# Autodesk Inventor assembly: Aimbot_Rev2
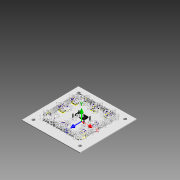
[picture p0: Inventor's stored thumbnail of the model, 180x180]
Saved by Autodesk Inventor 2015 (Build 190159000, 159)
## iProperties
Manager: Swagfish
Company: AntiWaseem Industries (AWI)
Created: 2014-05-17
Part Number: Aimbot_Rev2
Document SubType Name: Assembly
Designer: Joseph Varikooty
Mass: 2661.26 g
Surface Area: 7608.41 cm^2
Volume: 1160.78 cm^3
Density: 2.29266 g/cm^3
Author: Joseph Varikooty
Title: Aimbot Rev1.0
Subject: Rezzonating Swag
## Documents named in this file (97)
- X:\Dropbox\_School\AimBot\Aimbot_Rev2.iam
- X:\Dropbox\_School\AimBot\U-Channel Housing 4x2x12.ipt
- X:\Dropbox\_School\AimBot\HS-7940TH Servo.iam
- X:\Dropbox\_School\AimBot\Standard Servo Plate A (575112).ipt
- X:\Dropbox\_School\AimBot\Steel Ball Bearing (6383K245).iam
- X:\Dropbox\_School\AimBot\Turntable (1544T1).iam
- X:\Dropbox\_School\AimBot\Round Base A (585438).ipt
- X:\Dropbox\_School\AimBot\Bore Tube Clamp Hub (545340).ipt
- X:\Dropbox\_School\AimBot\Servo Hub - Tall (Hitec Standard) (ROB-12227).ipt
- X:\Dropbox\_School\AimBot\U Arms.ipt
- X:\Dropbox\_School\AimBot\Assembly1\Design Accelerator\Bolted Connection1.iam
- X:\Dropbox\_School\AimBot\Assembly1\Design Accelerator\Bolted Connection2.iam
- X:\Dropbox\_School\AimBot\Assembly1\Design Accelerator\Bolted Connection3.iam
- X:\Dropbox\_School\AimBot\Assembly1\Design Accelerator\Bolted Connection4.iam
- X:\Dropbox\_School\AimBot\Assembly1\Design Accelerator\Bolted Connection5.iam
- X:\Dropbox\_School\AimBot\Assembly1\Design Accelerator\Bolted Connection6.iam
- X:\Dropbox\_School\AimBot\Assembly1\Design Accelerator\Bolted Connection7.iam
- X:\Dropbox\_School\AimBot\Assembly1\Design Accelerator\Bolted Connection8.iam
- X:\Dropbox\_School\AimBot\Assembly1\Design Accelerator\Bolted Connection9.iam
- X:\Dropbox\_School\AimBot\Assembly1\Design Accelerator\Bolted Connection10.iam
- X:\Dropbox\_School\AimBot\Assembly1\Design Accelerator\Bolted Connection11.iam
- X:\Dropbox\_School\AimBot\Assembly1\Design Accelerator\Bolted Connection12.iam
- X:\Dropbox\_School\AimBot\Assembly1\Design Accelerator\Bolted Connection13.iam
- X:\Dropbox\_School\AimBot\64T Gear.ipt
- X:\Dropbox\_School\AimBot\32T Pinion Gear.ipt
- X:\Dropbox\_School\AimBot\Axail Rod.ipt
- X:\Dropbox\_School\AimBot\Spacer_ServoTilitBracketArm.ipt
- X:\Dropbox\_School\AimBot\Assembly1\Design Accelerator\Bolted Connection14.iam
- X:\Dropbox\_School\AimBot\Assembly1\Design Accelerator\Bolted Connection15.iam
- X:\Dropbox\_School\AimBot\Assembly1\Design Accelerator\Bolted Connection16.iam
- X:\Dropbox\_School\AimBot\Assembly1\Design Accelerator\Bolted Connection17.iam
- X:\Dropbox\_School\AimBot\Standoff_ServoTilitGearHub.ipt
- X:\Dropbox\_School\AimBot\Assembly1\Design Accelerator\Bolted Connection18.iam
- X:\Dropbox\_School\AimBot\Assembly1\Design Accelerator\Bolted Connection19.iam
- X:\Dropbox\_School\AimBot\Assembly1\Design Accelerator\Bolted Connection20.iam
- X:\Dropbox\_School\AimBot\Assembly1\Design Accelerator\Bolted Connection21.iam
- X:\Dropbox\_School\AimBot\Assembly1\Design Accelerator\Bolted Connection22.iam
- X:\Dropbox\_School\AimBot\Assembly1\Design Accelerator\Bolted Connection23.iam
- X:\Dropbox\_School\AimBot\Assembly1\Design Accelerator\Bolted Connection24.iam
- X:\Dropbox\_School\AimBot\Assembly1\Design Accelerator\Bolted Connection25.iam
- X:\Dropbox\_School\AimBot\Assembly1\Design Accelerator\Bolted Connection26.iam
- X:\Dropbox\_School\AimBot\Assembly1\Design Accelerator\Bolted Connection27.iam
- X:\Dropbox\_School\AimBot\Assembly1\Design Accelerator\Bolted Connection28.iam
- X:\Dropbox\_School\AimBot\Assembly1\Design Accelerator\Bolted Connection29.iam
- X:\Dropbox\_School\AimBot\Assembly1\Design Accelerator\Bolted Connection30.iam
- X:\Dropbox\_School\AimBot\Assembly1\Design Accelerator\Bolted Connection31.iam
- X:\Dropbox\_School\AimBot\Assembly1\Design Accelerator\Bolted Connection32.iam
- X:\Dropbox\_School\AimBot\Assembly1\Design Accelerator\Bolted Connection33.iam
- X:\Dropbox\_School\AimBot\Assembly1\Design Accelerator\Bolted Connection34.iam
- X:\Dropbox\_School\AimBot\Assembly1\Design Accelerator\Bolted Connection35.iam
- X:\Dropbox\_School\AimBot\Assembly1\Design Accelerator\Bolted Connection36.iam
- X:\Dropbox\_School\AimBot\Assembly1\Design Accelerator\Bolted Connection37.iam
- X:\Dropbox\_School\AimBot\Assembly1\Design Accelerator\Bolted Connection38.iam
- X:\Dropbox\_School\AimBot\Assembly1\Design Accelerator\Bolted Connection39.iam
- X:\Dropbox\_School\AimBot\Assembly1\Design Accelerator\Bolted Connection40.iam
- X:\Dropbox\_School\AimBot\Assembly1\Design Accelerator\Bolted Connection41.iam
- X:\Dropbox\_School\AimBot\Standoff_ServoPanBasePlate.ipt
- X:\Dropbox\_School\AimBot\SealWasher.ipt
- X:\Dropbox\_School\AimBot\Assembly1\Design Accelerator\Bolted Connection54.iam
- X:\Dropbox\_School\AimBot\Assembly1\Design Accelerator\Bolted Connection55.iam
- X:\Dropbox\_School\AimBot\Assembly1\Design Accelerator\Bolted Connection56.iam
- X:\Dropbox\_School\AimBot\Assembly1\Design Accelerator\Bolted Connection57.iam
- X:\Dropbox\_School\AimBot\Assembly1\Design Accelerator\Bolted Connection58.iam
- X:\Dropbox\_School\AimBot\Assembly1\Design Accelerator\Bolted Connection59.iam
- X:\Dropbox\_School\AimBot\Assembly1\Design Accelerator\Bolted Connection60.iam
- X:\Dropbox\_School\AimBot\Assembly1\Design Accelerator\Bolted Connection61.iam
- X:\Dropbox\_School\AimBot\Assembly1\Design Accelerator\Bolted Connection62.iam
- X:\Dropbox\_School\AimBot\Assembly1\Design Accelerator\Bolted Connection63.iam
- X:\Dropbox\_School\AimBot\Assembly1\Design Accelerator\Bolted Connection64.iam
- X:\Dropbox\_School\AimBot\Assembly1\Design Accelerator\Bolted Connection65.iam
- X:\Dropbox\_School\AimBot\Assembly1\Design Accelerator\Bolted Connection66.iam
- X:\Dropbox\_School\AimBot\ODROID-XU+E.ipt
- X:\Dropbox\_School\AimBot\Assembly1\Design Accelerator\Bolted Connection67.iam
- X:\Dropbox\_School\AimBot\Assembly1\Design Accelerator\Bolted Connection68.iam
- X:\Dropbox\_School\AimBot\Assembly1\Design Accelerator\Bolted Connection69.iam
- X:\Dropbox\_School\AimBot\Assembly1\Design Accelerator\Bolted Connection70.iam
- X:\Dropbox\_School\AimBot\Bracket (15275A53).ipt
- X:\Dropbox\_School\AimBot\Base_Master_Rev2.ipt
- X:\Dropbox\_School\AimBot\BottomBasePlate_Rev2.ipt
- X:\Dropbox\_School\AimBot\Bracket (15275A53)_LeftCut.ipt
- X:\Dropbox\_School\AimBot\Aimbot_Rev2\Design Accelerator\Bolted Connection1.iam
- X:\Dropbox\_School\AimBot\Aimbot_Rev2\Design Accelerator\Bolted Connection2.iam
- X:\Dropbox\_School\AimBot\Aimbot_Rev2\Design Accelerator\Bolted Connection3.iam
- X:\Dropbox\_School\AimBot\Aimbot_Rev2\Design Accelerator\Bolted Connection4.iam
- X:\Dropbox\_School\AimBot\Aimbot_Rev2\Design Accelerator\Bolted Connection5.iam
- X:\Dropbox\_School\AimBot\Aimbot_Rev2\Design Accelerator\Bolted Connection6.iam
- X:\Dropbox\_School\AimBot\Aimbot_Rev2\Design Accelerator\Bolted Connection7.iam
- X:\Dropbox\_School\AimBot\Aimbot_Rev2\Design Accelerator\Bolted Connection8.iam
- X:\Dropbox\_School\AimBot\Aimbot_Rev2\Design Accelerator\Bolted Connection9.iam
- X:\Dropbox\_School\AimBot\Aimbot_Rev2\Design Accelerator\Bolted Connection10.iam
- X:\Dropbox\_School\AimBot\Aimbot_Rev2\Design Accelerator\Bolted Connection11.iam
- X:\Dropbox\_School\AimBot\Aimbot_Rev2\Design Accelerator\Bolted Connection12.iam
- X:\Dropbox\_School\AimBot\Aimbot_Rev2\Design Accelerator\Bolted Connection13.iam
- X:\Dropbox\_School\AimBot\Aimbot_Rev2\Design Accelerator\Bolted Connection14.iam
- X:\Dropbox\_School\AimBot\Aimbot_Rev2\Design Accelerator\Bolted Connection15.iam
- X:\Dropbox\_School\AimBot\Aimbot_Rev2\Design Accelerator\Bolted Connection16.iam
- X:\Dropbox\_School\AimBot\Aimbot_Rev2\Design Accelerator\Bolted Connection17.iam
## Components (133 placed, 22 different names)
1. U-Channel Housing 4x2x12:1 — Mate:4, Mate:5, Mate:6, Mate:7, Mate:8, Mate:9, Mate:26, Mate:27, Mate:28, Mate:29, Mate:30, Mate:31, Mate:32, Mate:33, Mate:34, Mate:35, Mate:36, Mate:37, Mate:38, Mate:39, Mate:40, Mate:41, Mate:42, Mate:43
2. HS-7940TH Servo:1 [sub-assembly] — RemoveAfterScrews:1, RemoveAfterScrews:2, Mate:46, Mate:47, Mate:48, Mate:50, Mate:51, Mate:52, Mate:219, Mate:221, Mate:223, Mate:225
3. Standard Servo Plate A (575112):1 — RemoveAfterScrews:1, RemoveAfterScrews:2, Mate:51, Mate:61, Mate:63, Mate:65, Mate:67, Mate:56, Mate:54, Mate:220, Mate:222, Mate:224, Mate:226
4. Steel Ball Bearing (6383K245):1 [sub-assembly] — Rigid:1, Cylindrical:2
5. Steel Ball Bearing (6383K245):2 [sub-assembly] — Rigid:2, Cylindrical:1, Flush:3
6. Turntable (1544T1):1 [sub-assembly] — Mate:10, Mate:11, Mate:12, Mate:136, Mate:137, Mate:138, Mate:139, Mate:140, Mate:141, Mate:143, Mate:145, Mate:147
7. Round Base A (585438):1 — Mate:21, BaseHub:22, BaseHub:23, BaseHub:24, BaseHub:25, BaseArm:97, BaseArm:98, BaseArm:99, BaseArm:100, Mate:101, Mate:109, Mate:111, Mate:113, Mate:115, Mate:117, Mate:119, Mate:121, Mate:123, Mate:125, Mate:127, Mate:129, Mate:131
8. Bore Tube Clamp Hub (545340):1 — Mate:7, Mate:8, Mate:9, Mate:45, Mate:69, Mate:70, Mate:71, Mate:72, Mate:73, Mate:74, Mate:75, Mate:76, Mate:80, Mate:89, Mate:90, Mate:91, Mate:92
9. Bore Tube Clamp Hub (545340):2 — Mate:4, Mate:5, Mate:6, Mate:44, Mate:93, Mate:94, Mate:95, Mate:96
10. Servo Hub - Tall (Hitec Standard) (ROB-12227):2 — Mate:21, BaseHub:22, BaseHub:23, BaseHub:24, BaseHub:25, Mate:134, Mate:135
11. HS-7940TH Servo:2 [sub-assembly] — Mate:3, Mate:132, Mate:133, Mate:134, Mate:135, Mate:227, Mate:229, Mate:231, Mate:233, Mate:235
12. Standard Servo Plate A (575112):2 — Mate:3, Mate:132, Mate:133, Angle:1, Mate:204, Mate:205, Mate:206, Mate:207, Mate:208, Mate:209, Mate:210, Mate:211, Mate:213, Mate:215, Mate:217, Mate:228, Mate:230, Mate:232, Mate:234, Mate:236
13. U Arms:1 — Rigid:1, Rigid:2, Mate:10, Mate:11, Mate:12, Mate:13, Mate:14, Mate:15, Mate:16, Mate:17, Mate:18, Mate:19, Mate:20, Mate:50, Mate:52, Mate:55, Mate:57, Mate:58, Mate:59, Mate:60, Mate:62, Mate:64, Mate:66, Mate:68, BaseArm:97, BaseArm:98, BaseArm:99, BaseArm:100, Mate:101, Mate:108, Mate:110, Mate:112, Mate:114, Mate:116, Mate:118, Mate:120, Mate:122, Mate:124, Mate:126, Mate:128, Mate:130
14. Bolted Connection:1 [sub-assembly] — Mate:13, Mate:14
15. Bolted Connection:2 [sub-assembly] — Mate:15, Mate:16
16. Bolted Connection:3 [sub-assembly] — Mate:17, Mate:18
17. Bolted Connection:4 [sub-assembly] — Mate:19, Mate:20
18. Bolted Connection:5 [sub-assembly] — Mate:26, Mate:27
19. Bolted Connection:6 [sub-assembly] — Mate:28, Mate:29
20. Bolted Connection:7 [sub-assembly] — Mate:30, Mate:31
21. Bolted Connection:8 [sub-assembly] — Mate:32, Mate:33
22. Bolted Connection:9 [sub-assembly] — Mate:34, Mate:35
23. Bolted Connection:10 [sub-assembly] — Mate:36, Mate:37
24. Bolted Connection:11 [sub-assembly] — Mate:38, Mate:39
25. Bolted Connection:12 [sub-assembly] — Mate:40, Mate:41
26. Bolted Connection:13 [sub-assembly] — Mate:42, Mate:43
27. 64T Gear:1 — Cylindrical:3, Rotation:1, Mate:79, Mate:80, Mate:81, Mate:82, Mate:83, Mate:84, Mate:85, Mate:86, Mate:87, Mate:88
28. 32T Pinion Gear:1 — Mate:46, Mate:47, Mate:48, Mate:49, Flush:2, Rotation:1
29. Axail Rod:1 — Cylindrical:1, Cylindrical:3, Mate:45, Mate:49, Flush:3
30. Axail Rod:2 — Cylindrical:2, Mate:44
31. Spacer_ServoTilitBracketArm:1 — Mate:53, Mate:54
32. Spacer_ServoTilitBracketArm:2 — Mate:55, Mate:56
33. Spacer_ServoTilitBracketArm:3 — Mate:57, Mate:58
34. Spacer_ServoTilitBracketArm:4 — Mate:59, Mate:60
35. Bolted Connection:14 [sub-assembly] — Mate:61, Mate:62
36. Bolted Connection:15 [sub-assembly] — Mate:63, Mate:64
37. Bolted Connection:16 [sub-assembly] — Mate:65, Mate:66
38. Bolted Connection:17 [sub-assembly] — Mate:67, Mate:68, Mate:53
39. Standoff_ServoTilitGearHub:1 — Mate:71, Mate:76, Mate:79
40. Standoff_ServoTilitGearHub:2 — Mate:70, Mate:74
41. Standoff_ServoTilitGearHub:3 — Mate:72, Mate:75
42. Standoff_ServoTilitGearHub:4 — Mate:69, Mate:73
43. Bolted Connection:18 [sub-assembly] — Mate:81, Mate:82
44. Bolted Connection:19 [sub-assembly] — Mate:83, Mate:84
45. Bolted Connection:20 [sub-assembly] — Mate:85, Mate:86
46. Bolted Connection:21 [sub-assembly] — Mate:87, Mate:88
47. Bolted Connection:22 [sub-assembly] — Mate:89, Mate:90
48. Bolted Connection:23 [sub-assembly] — Mate:91, Mate:92
49. Bolted Connection:24 [sub-assembly] — Mate:93, Mate:94
50. Bolted Connection:25 [sub-assembly] — Mate:95, Mate:96
51. Bolted Connection:26 [sub-assembly] — Mate:114, Mate:115
52. Bolted Connection:27 [sub-assembly] — Mate:112, Mate:113
53. Bolted Connection:28 [sub-assembly] — Mate:110, Mate:111
54. Bolted Connection:29 [sub-assembly] — Mate:108, Mate:109
55. Bolted Connection:30 [sub-assembly] — Mate:116, Mate:117
56. Bolted Connection:31 [sub-assembly] — Mate:118, Mate:119
57. Bolted Connection:32 [sub-assembly] — Mate:120, Mate:121
58. Bolted Connection:33 [sub-assembly] — Mate:122, Mate:123
59. Bolted Connection:34 [sub-assembly] — Mate:124, Mate:125
60. Bolted Connection:35 [sub-assembly] — Mate:126, Mate:127
61. Bolted Connection:36 [sub-assembly] — Mate:128, Mate:129
62. Bolted Connection:37 [sub-assembly] — Mate:130, Mate:131
63. BottomBasePlate_Rev2:1 — Mate:180, Mate:181, Mate:186, Mate:187, Mate:192, Mate:193, Mate:198, Mate:199, Angle:2, Mate:239, Mate:240, Mate:241, Mate:242, Mate:243, Mate:244, Mate:245, Mate:246, Mate:250, Mate:251, Mate:252, Mate:259, Mate:260, Mate:261, Mate:266, Mate:269, Mate:272, Mate:275, Mate:278, Mate:281, Mate:283, Mate:284, Mate:285, Mate:286, Mate:287, Mate:288, Mate:289, Mate:290, Mate:291, Mate:292, Mate:293, Mate:294, Mate:295, Mate:296, Mate:297, Mate:298, Mate:299, Mate:300, Mate:301, Mate:302, Mate:303, Mate:304
64. Base_Master_Rev2:1 — Mate:136, Mate:137, Mate:138, Mate:139, Mate:140, Mate:142, Mate:144, Mate:146, Mate:148, Angle:1, Mate:247, Mate:248, Mate:249, Mate:253, Mate:254, Mate:255, Mate:256, Mate:257, Mate:258, Mate:262, Mate:263, Mate:264, Mate:265, Mate:267, Mate:268, Mate:270, Mate:271, Mate:273, Mate:274, Mate:276, Mate:277, Mate:279, Mate:280, Mate:282, Mate:305, Mate:306, Mate:307, Mate:308, Mate:309, Mate:310, Mate:311, Mate:312, Mate:313, Mate:314, Mate:315, Mate:316
65. Bolted Connection:38 [sub-assembly] — Mate:141, Mate:142
66. Bolted Connection:39 [sub-assembly] — Mate:143, Mate:144
67. Bolted Connection:40 [sub-assembly] — Mate:145, Mate:146
68. Bolted Connection:41 [sub-assembly] — Mate:147, Mate:148
69. Standoff_ServoPanBasePlate:1 — Mate:200, Mate:205, Mate:207, Mate:214
70. Standoff_ServoPanBasePlate:2 — Mate:201, Mate:206, Mate:209, Mate:212
71. Standoff_ServoPanBasePlate:3 — Mate:203, Mate:210, Mate:216
72. Standoff_ServoPanBasePlate:4 — Mate:202, Mate:204, Mate:208, Mate:218
73. SealWasher:1 — Mate:189, Mate:191, Mate:202
74. SealWasher:2 — Mate:188, Mate:189, Mate:190, Mate:191
75. SealWasher:3 — Mate:188, Mate:190, Mate:192, Mate:193
76. SealWasher:4 — Mate:183, Mate:185, Mate:203
77. SealWasher:5 — Mate:182, Mate:183, Mate:184, Mate:186, Mate:187
78. SealWasher:6 — Mate:182, Mate:184, Mate:185
79. SealWasher:7 — Mate:177, Mate:178, Mate:201
80. SealWasher:8 — Mate:176, Mate:177, Mate:178, Mate:179
81. SealWasher:9 — Mate:176, Mate:179, Mate:180, Mate:181
82. SealWasher:10 — Mate:195, Mate:197, Mate:200
83. SealWasher:11 — Mate:194, Mate:195, Mate:196, Mate:197
84. SealWasher:12 — Mate:194, Mate:196, Mate:198, Mate:199
85. Bolted Connection:54 [sub-assembly] — Mate:211, Mate:212
86. Bolted Connection:55 [sub-assembly] — Mate:213, Mate:214
87. Bolted Connection:56 [sub-assembly] — Mate:215, Mate:216
88. Bolted Connection:57 [sub-assembly] — Mate:217, Mate:218
89. Bolted Connection:58 [sub-assembly] — Mate:219, Mate:220
90. Bolted Connection:59 [sub-assembly] — Mate:221, Mate:222
91. Bolted Connection:60 [sub-assembly] — Mate:223, Mate:224
92. Bolted Connection:61 [sub-assembly] — Mate:225, Mate:226
93. Bolted Connection:62 [sub-assembly] — Mate:227, Mate:228
94. Bolted Connection:63 [sub-assembly] — Mate:229, Mate:230
95. Bolted Connection:64 [sub-assembly] — Mate:231, Mate:232
96. Bolted Connection:65 [sub-assembly] — Mate:233, Mate:234
97. Bolted Connection:66 [sub-assembly] — Mate:235, Mate:236
98. ODROID-XU+E:1 — Angle:2
99. Bolted Connection:67 [sub-assembly] — Mate:241, Mate:242
100. Bolted Connection:68 [sub-assembly] — Mate:239, Mate:240
101. Bolted Connection:69 [sub-assembly] — Mate:243, Mate:244
102. Bolted Connection:70 [sub-assembly] — Mate:245, Mate:246
103. Bracket (15275A53):1 — Mate:249, Mate:252, Mate:253
104. Bracket (15275A53)_LeftCut:2 — Mate:247, Mate:250, Mate:255
105. Bracket (15275A53):3 — Mate:248, Mate:251, Mate:254
106. Bracket (15275A53)_LeftCut:3 — Mate:258, Mate:259, Mate:262
107. Bracket (15275A53):5 — Mate:256, Mate:261, Mate:264
108. Bracket (15275A53):6 — Mate:257, Mate:260, Mate:263
109. Bracket (15275A53):7 — Mate:268, Mate:269, Mate:270
110. Bracket (15275A53):8
111. Bracket (15275A53)_LeftCut:1 — Mate:265, Mate:266, Mate:267
112. Bracket (15275A53):9 — Mate:271, Mate:272, Mate:273
113. Bracket (15275A53):10
114. Bracket (15275A53):11 — Mate:274, Mate:275, Mate:276
115. Bracket (15275A53)_LeftCut:4 — Mate:280, Mate:281, Mate:282
116. Bracket (15275A53):13 — Mate:277, Mate:278, Mate:279
117. Bolted Connection:71 [sub-assembly] — Mate:283, Mate:284
118. Bolted Connection:72 [sub-assembly] — Mate:285, Mate:286
119. Bolted Connection:73 [sub-assembly] — Mate:287, Mate:288
120. Bolted Connection:74 [sub-assembly] — Mate:289, Mate:290
121. Bolted Connection:75 [sub-assembly] — Mate:291, Mate:292
122. Bolted Connection:76 [sub-assembly] — Mate:293, Mate:294
123. Bolted Connection:77 [sub-assembly] — Mate:295, Mate:296
124. Bolted Connection:78 [sub-assembly] — Mate:297, Mate:298
125. Bolted Connection:79 [sub-assembly] — Mate:299, Mate:300
126. Bolted Connection:80 [sub-assembly] — Mate:301, Mate:302
127. Bolted Connection:81 [sub-assembly] — Mate:303, Mate:304
128. Bolted Connection:82 [sub-assembly] — Mate:305, Mate:306
129. Bolted Connection:83 [sub-assembly] — Mate:307, Mate:308
130. Bolted Connection:84 [sub-assembly] — Mate:309, Mate:310
131. Bolted Connection:85 [sub-assembly] — Mate:311, Mate:312
132. Bolted Connection:86 [sub-assembly] — Mate:313, Mate:314
133. Bolted Connection:87 [sub-assembly] — Mate:315, Mate:316
## Relationships (289: Mate 279, CylindricalJoint 3, WeldJoint 2, Flush 2, Angle 2, RelateRotation 1)
- RemoveAfterScrews:1 [Mate]: HS-7940TH Servo:1 ↔ Standard Servo Plate A (575112):1
- RemoveAfterScrews:2 [Mate] (0.1651 mm): HS-7940TH Servo:1 ↔ Standard Servo Plate A (575112):1
- Mate:3 (0.1651 mm): HS-7940TH Servo:2 ↔ Standard Servo Plate A (575112):2
- Rigid:1 [WeldJoint]: Steel Ball Bearing (6383K245):1 ↔ U Arms:1
- Rigid:2 [WeldJoint]: Steel Ball Bearing (6383K245):2 ↔ U Arms:1
- Mate:4: U-Channel Housing 4x2x12:1 ↔ Bore Tube Clamp Hub (545340):2
- Mate:5: U-Channel Housing 4x2x12:1 ↔ Bore Tube Clamp Hub (545340):2
- Mate:6: U-Channel Housing 4x2x12:1 ↔ Bore Tube Clamp Hub (545340):2
- Mate:7: U-Channel Housing 4x2x12:1 ↔ Bore Tube Clamp Hub (545340):1
- Mate:8: U-Channel Housing 4x2x12:1 ↔ Bore Tube Clamp Hub (545340):1
- Mate:9: U-Channel Housing 4x2x12:1 ↔ Bore Tube Clamp Hub (545340):1
- Mate:10: Turntable (1544T1):1 ↔ U Arms:1
- Mate:11: Turntable (1544T1):1 ↔ U Arms:1
- Mate:12: Turntable (1544T1):1 ↔ U Arms:1
- Mate:13: U Arms:1 ↔ Bolted Connection:1
- Mate:14: U Arms:1 ↔ Bolted Connection:1
- Mate:15: U Arms:1 ↔ Bolted Connection:2
- Mate:16: U Arms:1 ↔ Bolted Connection:2
- Mate:17: U Arms:1 ↔ Bolted Connection:3
- Mate:18: U Arms:1 ↔ Bolted Connection:3
- Mate:19: U Arms:1 ↔ Bolted Connection:4
- Mate:20: U Arms:1 ↔ Bolted Connection:4
- Mate:21: Round Base A (585438):1 ↔ Servo Hub - Tall (Hitec Standard) (ROB-12227):2
- BaseHub:22 [Mate]: Round Base A (585438):1 ↔ Servo Hub - Tall (Hitec Standard) (ROB-12227):2
- BaseHub:23 [Mate]: Round Base A (585438):1 ↔ Servo Hub - Tall (Hitec Standard) (ROB-12227):2
- BaseHub:24 [Mate]: Round Base A (585438):1 ↔ Servo Hub - Tall (Hitec Standard) (ROB-12227):2
- BaseHub:25 [Mate]: Round Base A (585438):1 ↔ Servo Hub - Tall (Hitec Standard) (ROB-12227):2
- Mate:26: U-Channel Housing 4x2x12:1 ↔ Bolted Connection:5
- Mate:27: U-Channel Housing 4x2x12:1 ↔ Bolted Connection:5
- Mate:28: U-Channel Housing 4x2x12:1 ↔ Bolted Connection:6
- Mate:29: U-Channel Housing 4x2x12:1 ↔ Bolted Connection:6
- Mate:30: U-Channel Housing 4x2x12:1 ↔ Bolted Connection:7
- Mate:31: U-Channel Housing 4x2x12:1 ↔ Bolted Connection:7
- Mate:32: U-Channel Housing 4x2x12:1 ↔ Bolted Connection:8
- Mate:33: U-Channel Housing 4x2x12:1 ↔ Bolted Connection:8
- Mate:34: U-Channel Housing 4x2x12:1 ↔ Bolted Connection:9
- Mate:35: U-Channel Housing 4x2x12:1 ↔ Bolted Connection:9
- Mate:36: U-Channel Housing 4x2x12:1 ↔ Bolted Connection:10
- Mate:37: U-Channel Housing 4x2x12:1 ↔ Bolted Connection:10
- Mate:38: U-Channel Housing 4x2x12:1 ↔ Bolted Connection:11
- Mate:39: U-Channel Housing 4x2x12:1 ↔ Bolted Connection:11
- Mate:40: U-Channel Housing 4x2x12:1 ↔ Bolted Connection:12
- Mate:41: U-Channel Housing 4x2x12:1 ↔ Bolted Connection:12
- Mate:42: U-Channel Housing 4x2x12:1 ↔ Bolted Connection:13
- Mate:43: U-Channel Housing 4x2x12:1 ↔ Bolted Connection:13
- Cylindrical:1: Steel Ball Bearing (6383K245):2 ↔ Axail Rod:1
- Cylindrical:2: Steel Ball Bearing (6383K245):1 ↔ Axail Rod:2
- Cylindrical:3: 64T Gear:1 ↔ Axail Rod:1
- Mate:44: Bore Tube Clamp Hub (545340):2 ↔ Axail Rod:2
- Mate:45: Bore Tube Clamp Hub (545340):1 ↔ Axail Rod:1
- Mate:46: HS-7940TH Servo:1 ↔ 32T Pinion Gear:1
- Mate:47 (3.048 mm): HS-7940TH Servo:1 ↔ 32T Pinion Gear:1
- Mate:48: HS-7940TH Servo:1 ↔ 32T Pinion Gear:1
- Mate:49 (38.1 mm): 32T Pinion Gear:1 ↔ Axail Rod:1
- Flush:2: 32T Pinion Gear:1
- Rotation:1 [RelateRotation] (2 ul): 64T Gear:1 ↔ 32T Pinion Gear:1
- Mate:50: HS-7940TH Servo:1 ↔ U Arms:1
- Mate:51 (0.8255 mm): HS-7940TH Servo:1 ↔ Standard Servo Plate A (575112):1
- Mate:52: HS-7940TH Servo:1 ↔ U Arms:1
- Mate:53: Spacer_ServoTilitBracketArm:1 ↔ Bolted Connection:17
- Mate:54: Standard Servo Plate A (575112):1 ↔ Spacer_ServoTilitBracketArm:1
- Mate:55: U Arms:1 ↔ Spacer_ServoTilitBracketArm:2
- Mate:56: Standard Servo Plate A (575112):1 ↔ Spacer_ServoTilitBracketArm:2
- Mate:57: U Arms:1 ↔ Spacer_ServoTilitBracketArm:3
- Mate:58: U Arms:1 ↔ Spacer_ServoTilitBracketArm:3
- Mate:59: U Arms:1 ↔ Spacer_ServoTilitBracketArm:4
- Mate:60: U Arms:1 ↔ Spacer_ServoTilitBracketArm:4
- Mate:61: Standard Servo Plate A (575112):1 ↔ Bolted Connection:14
- Mate:62: U Arms:1 ↔ Bolted Connection:14
- Mate:63: Standard Servo Plate A (575112):1 ↔ Bolted Connection:15
- Mate:64: U Arms:1 ↔ Bolted Connection:15
- Mate:65: Standard Servo Plate A (575112):1 ↔ Bolted Connection:16
- Mate:66: U Arms:1 ↔ Bolted Connection:16
- Mate:67: Standard Servo Plate A (575112):1 ↔ Bolted Connection:17
- Mate:68: U Arms:1 ↔ Bolted Connection:17
- Mate:69: Bore Tube Clamp Hub (545340):1 ↔ Standoff_ServoTilitGearHub:4
- Mate:70: Bore Tube Clamp Hub (545340):1 ↔ Standoff_ServoTilitGearHub:2
- Mate:71: Bore Tube Clamp Hub (545340):1 ↔ Standoff_ServoTilitGearHub:1
- Mate:72: Bore Tube Clamp Hub (545340):1 ↔ Standoff_ServoTilitGearHub:3
- Mate:73: Bore Tube Clamp Hub (545340):1 ↔ Standoff_ServoTilitGearHub:4
- Mate:74: Bore Tube Clamp Hub (545340):1 ↔ Standoff_ServoTilitGearHub:2
- Mate:75: Bore Tube Clamp Hub (545340):1 ↔ Standoff_ServoTilitGearHub:3
- Mate:76: Bore Tube Clamp Hub (545340):1 ↔ Standoff_ServoTilitGearHub:1
- Mate:79: 64T Gear:1 ↔ Standoff_ServoTilitGearHub:1
- Mate:80: Bore Tube Clamp Hub (545340):1 ↔ 64T Gear:1
- Mate:81: 64T Gear:1 ↔ Bolted Connection:18
- Mate:82: 64T Gear:1 ↔ Bolted Connection:18
- Mate:83: 64T Gear:1 ↔ Bolted Connection:19
- Mate:84: 64T Gear:1 ↔ Bolted Connection:19
- Mate:85: 64T Gear:1 ↔ Bolted Connection:20
- Mate:86: 64T Gear:1 ↔ Bolted Connection:20
- Mate:87: 64T Gear:1 ↔ Bolted Connection:21
- Mate:88: 64T Gear:1 ↔ Bolted Connection:21
- Flush:3 (-1.524 mm): Steel Ball Bearing (6383K245):2 ↔ Axail Rod:1
- Mate:89: Bore Tube Clamp Hub (545340):1 ↔ Bolted Connection:22
- Mate:90: Bore Tube Clamp Hub (545340):1 ↔ Bolted Connection:22
- Mate:91: Bore Tube Clamp Hub (545340):1 ↔ Bolted Connection:23
- Mate:92: Bore Tube Clamp Hub (545340):1 ↔ Bolted Connection:23
- Mate:93: Bore Tube Clamp Hub (545340):2 ↔ Bolted Connection:24
- Mate:94: Bore Tube Clamp Hub (545340):2 ↔ Bolted Connection:24
- Mate:95: Bore Tube Clamp Hub (545340):2 ↔ Bolted Connection:25
- Mate:96: Bore Tube Clamp Hub (545340):2 ↔ Bolted Connection:25
- BaseArm:97 [Mate]: Round Base A (585438):1 ↔ U Arms:1
- BaseArm:98 [Mate]: Round Base A (585438):1 ↔ U Arms:1
- BaseArm:99 [Mate]: Round Base A (585438):1 ↔ U Arms:1
- BaseArm:100 [Mate]: Round Base A (585438):1 ↔ U Arms:1
- Mate:101: Round Base A (585438):1 ↔ U Arms:1
- Mate:108: U Arms:1 ↔ Bolted Connection:29
- Mate:109: Round Base A (585438):1 ↔ Bolted Connection:29
- Mate:110: U Arms:1 ↔ Bolted Connection:28
- Mate:111: Round Base A (585438):1 ↔ Bolted Connection:28
- Mate:112: U Arms:1 ↔ Bolted Connection:27
- Mate:113: Round Base A (585438):1 ↔ Bolted Connection:27
- Mate:114: U Arms:1 ↔ Bolted Connection:26
- Mate:115: Round Base A (585438):1 ↔ Bolted Connection:26
- Mate:116: U Arms:1 ↔ Bolted Connection:30
- Mate:117: Round Base A (585438):1 ↔ Bolted Connection:30
- Mate:118: U Arms:1 ↔ Bolted Connection:31
- Mate:119: Round Base A (585438):1 ↔ Bolted Connection:31
- Mate:120: U Arms:1 ↔ Bolted Connection:32
- Mate:121: Round Base A (585438):1 ↔ Bolted Connection:32
- Mate:122: U Arms:1 ↔ Bolted Connection:33
- Mate:123: Round Base A (585438):1 ↔ Bolted Connection:33
- Mate:124: U Arms:1 ↔ Bolted Connection:34
- Mate:125: Round Base A (585438):1 ↔ Bolted Connection:34
- Mate:126: U Arms:1 ↔ Bolted Connection:35
- Mate:127: Round Base A (585438):1 ↔ Bolted Connection:35
- Mate:128: U Arms:1 ↔ Bolted Connection:36
- Mate:129: Round Base A (585438):1 ↔ Bolted Connection:36
- Mate:130: U Arms:1 ↔ Bolted Connection:37
- Mate:131: Round Base A (585438):1 ↔ Bolted Connection:37
- Mate:132 (0.8255 mm): HS-7940TH Servo:2 ↔ Standard Servo Plate A (575112):2
- Mate:133: HS-7940TH Servo:2 ↔ Standard Servo Plate A (575112):2
- Mate:134: Servo Hub - Tall (Hitec Standard) (ROB-12227):2 ↔ HS-7940TH Servo:2
- Mate:135 (3.048 mm): Servo Hub - Tall (Hitec Standard) (ROB-12227):2 ↔ HS-7940TH Servo:2
- Mate:136: Turntable (1544T1):1 ↔ Base_Master_Rev2:1
- Mate:137: Turntable (1544T1):1 ↔ Base_Master_Rev2:1
- Mate:138: Turntable (1544T1):1 ↔ Base_Master_Rev2:1
- Mate:139: Turntable (1544T1):1 ↔ Base_Master_Rev2:1
- Mate:140: Turntable (1544T1):1 ↔ Base_Master_Rev2:1
- Mate:141: Turntable (1544T1):1 ↔ Bolted Connection:38
- Mate:142: Base_Master_Rev2:1 ↔ Bolted Connection:38
- Mate:143: Turntable (1544T1):1 ↔ Bolted Connection:39
- Mate:144: Base_Master_Rev2:1 ↔ Bolted Connection:39
- Mate:145: Turntable (1544T1):1 ↔ Bolted Connection:40
- Mate:146: Base_Master_Rev2:1 ↔ Bolted Connection:40
- Mate:147: Turntable (1544T1):1 ↔ Bolted Connection:41
- Mate:148: Base_Master_Rev2:1 ↔ Bolted Connection:41
- Mate:176: SealWasher:8 ↔ SealWasher:9
- Mate:177: SealWasher:7 ↔ SealWasher:8
- Mate:178 (0.254 mm): SealWasher:7 ↔ SealWasher:8
- Mate:179 (0.254 mm): SealWasher:8 ↔ SealWasher:9
- Mate:180: BottomBasePlate_Rev2:1 ↔ SealWasher:9
- Mate:181 (0.127 mm): BottomBasePlate_Rev2:1 ↔ SealWasher:9
- Mate:182: SealWasher:5 ↔ SealWasher:6
- Mate:183: SealWasher:4 ↔ SealWasher:5
- Mate:184 (0.254 mm): SealWasher:5 ↔ SealWasher:6
- Mate:185 (0.254 mm): SealWasher:4 ↔ SealWasher:6
- Mate:186: BottomBasePlate_Rev2:1 ↔ SealWasher:5
- Mate:187 (0.127 mm): BottomBasePlate_Rev2:1 ↔ SealWasher:5
- Mate:188: SealWasher:2 ↔ SealWasher:3
- Mate:189: SealWasher:1 ↔ SealWasher:2
- Mate:190 (0.254 mm): SealWasher:2 ↔ SealWasher:3
- Mate:191 (0.254 mm): SealWasher:1 ↔ SealWasher:2
- Mate:192: BottomBasePlate_Rev2:1 ↔ SealWasher:3
- Mate:193 (0.127 mm): BottomBasePlate_Rev2:1 ↔ SealWasher:3
- Mate:194: SealWasher:11 ↔ SealWasher:12
- Mate:195: SealWasher:10 ↔ SealWasher:11
- Mate:196 (0.254 mm): SealWasher:11 ↔ SealWasher:12
- Mate:197 (0.254 mm): SealWasher:10 ↔ SealWasher:11
- Mate:198: BottomBasePlate_Rev2:1 ↔ SealWasher:12
- Mate:199 (0.127 mm): BottomBasePlate_Rev2:1 ↔ SealWasher:12
- Mate:200: Standoff_ServoPanBasePlate:1 ↔ SealWasher:10
- Mate:201: Standoff_ServoPanBasePlate:2 ↔ SealWasher:7
- Mate:202: Standoff_ServoPanBasePlate:4 ↔ SealWasher:1
- Mate:203: Standoff_ServoPanBasePlate:3 ↔ SealWasher:4
- Angle:1 (180 deg): Standard Servo Plate A (575112):2 ↔ Base_Master_Rev2:1
- Mate:204: Standard Servo Plate A (575112):2 ↔ Standoff_ServoPanBasePlate:4
- Mate:205: Standard Servo Plate A (575112):2 ↔ Standoff_ServoPanBasePlate:1
- Mate:206: Standard Servo Plate A (575112):2 ↔ Standoff_ServoPanBasePlate:2
- Mate:207: Standard Servo Plate A (575112):2 ↔ Standoff_ServoPanBasePlate:1
- Mate:208: Standard Servo Plate A (575112):2 ↔ Standoff_ServoPanBasePlate:4
- Mate:209: Standard Servo Plate A (575112):2 ↔ Standoff_ServoPanBasePlate:2
- Mate:210: Standard Servo Plate A (575112):2 ↔ Standoff_ServoPanBasePlate:3
- Mate:211: Standard Servo Plate A (575112):2 ↔ Bolted Connection:54
- Mate:212: Standoff_ServoPanBasePlate:2 ↔ Bolted Connection:54
- Mate:213: Standard Servo Plate A (575112):2 ↔ Bolted Connection:55
- Mate:214: Standoff_ServoPanBasePlate:1 ↔ Bolted Connection:55
- Mate:215: Standard Servo Plate A (575112):2 ↔ Bolted Connection:56
- Mate:216: Standoff_ServoPanBasePlate:3 ↔ Bolted Connection:56
- Mate:217: Standard Servo Plate A (575112):2 ↔ Bolted Connection:57
- Mate:218: Standoff_ServoPanBasePlate:4 ↔ Bolted Connection:57
- Mate:219: HS-7940TH Servo:1 ↔ Bolted Connection:58
- Mate:220: Standard Servo Plate A (575112):1 ↔ Bolted Connection:58
- Mate:221: HS-7940TH Servo:1 ↔ Bolted Connection:59
- Mate:222: Standard Servo Plate A (575112):1 ↔ Bolted Connection:59
- Mate:223: HS-7940TH Servo:1 ↔ Bolted Connection:60
- Mate:224: Standard Servo Plate A (575112):1 ↔ Bolted Connection:60
- Mate:225: HS-7940TH Servo:1 ↔ Bolted Connection:61
- Mate:226: Standard Servo Plate A (575112):1 ↔ Bolted Connection:61
- Mate:227: HS-7940TH Servo:2 ↔ Bolted Connection:62
- Mate:228: Standard Servo Plate A (575112):2 ↔ Bolted Connection:62
- Mate:229: HS-7940TH Servo:2 ↔ Bolted Connection:63
- Mate:230: Standard Servo Plate A (575112):2 ↔ Bolted Connection:63
- Mate:231: HS-7940TH Servo:2 ↔ Bolted Connection:64
- Mate:232: Standard Servo Plate A (575112):2 ↔ Bolted Connection:64
- Mate:233: HS-7940TH Servo:2 ↔ Bolted Connection:65
- Mate:234: Standard Servo Plate A (575112):2 ↔ Bolted Connection:65
- Mate:235: HS-7940TH Servo:2 ↔ Bolted Connection:66
- Mate:236: Standard Servo Plate A (575112):2 ↔ Bolted Connection:66
- Angle:2 (225 deg): BottomBasePlate_Rev2:1 ↔ ODROID-XU+E:1
- Mate:239: BottomBasePlate_Rev2:1 ↔ Bolted Connection:68
- Mate:240: BottomBasePlate_Rev2:1 ↔ Bolted Connection:68
- Mate:241: BottomBasePlate_Rev2:1 ↔ Bolted Connection:67
- Mate:242: BottomBasePlate_Rev2:1 ↔ Bolted Connection:67
- Mate:243: BottomBasePlate_Rev2:1 ↔ Bolted Connection:69
- Mate:244: BottomBasePlate_Rev2:1 ↔ Bolted Connection:69
- Mate:245: BottomBasePlate_Rev2:1 ↔ Bolted Connection:70
- Mate:246: BottomBasePlate_Rev2:1 ↔ Bolted Connection:70
- Mate:247: Base_Master_Rev2:1 ↔ Bracket (15275A53)_LeftCut:2
- Mate:248: Base_Master_Rev2:1 ↔ Bracket (15275A53):3
- Mate:249: Base_Master_Rev2:1 ↔ Bracket (15275A53):1
- Mate:250: BottomBasePlate_Rev2:1 ↔ Bracket (15275A53)_LeftCut:2
- Mate:251: BottomBasePlate_Rev2:1 ↔ Bracket (15275A53):3
- Mate:252: BottomBasePlate_Rev2:1 ↔ Bracket (15275A53):1
- Mate:253: Base_Master_Rev2:1 ↔ Bracket (15275A53):1
- Mate:254: Base_Master_Rev2:1 ↔ Bracket (15275A53):3
- Mate:255: Base_Master_Rev2:1 ↔ Bracket (15275A53)_LeftCut:2
- Mate:256: Base_Master_Rev2:1 ↔ Bracket (15275A53):5
- Mate:257: Base_Master_Rev2:1 ↔ Bracket (15275A53):6
- Mate:258: Base_Master_Rev2:1 ↔ Bracket (15275A53)_LeftCut:3
- Mate:259: BottomBasePlate_Rev2:1 ↔ Bracket (15275A53)_LeftCut:3
- Mate:260: BottomBasePlate_Rev2:1 ↔ Bracket (15275A53):6
- Mate:261: BottomBasePlate_Rev2:1 ↔ Bracket (15275A53):5
- Mate:262: Base_Master_Rev2:1 ↔ Bracket (15275A53)_LeftCut:3
- Mate:263: Base_Master_Rev2:1 ↔ Bracket (15275A53):6
- Mate:264: Base_Master_Rev2:1 ↔ Bracket (15275A53):5
- Mate:265: Base_Master_Rev2:1 ↔ Bracket (15275A53)_LeftCut:1
- Mate:266: BottomBasePlate_Rev2:1 ↔ Bracket (15275A53)_LeftCut:1
- Mate:267: Base_Master_Rev2:1 ↔ Bracket (15275A53)_LeftCut:1
- Mate:268: Base_Master_Rev2:1 ↔ Bracket (15275A53):7
- Mate:269: BottomBasePlate_Rev2:1 ↔ Bracket (15275A53):7
- Mate:270: Base_Master_Rev2:1 ↔ Bracket (15275A53):7
- Mate:271: Base_Master_Rev2:1 ↔ Bracket (15275A53):9
- Mate:272: BottomBasePlate_Rev2:1 ↔ Bracket (15275A53):9
- Mate:273: Base_Master_Rev2:1 ↔ Bracket (15275A53):9
- Mate:274: Base_Master_Rev2:1 ↔ Bracket (15275A53):11
- Mate:275: BottomBasePlate_Rev2:1 ↔ Bracket (15275A53):11
- Mate:276: Base_Master_Rev2:1 ↔ Bracket (15275A53):11
- Mate:277: Base_Master_Rev2:1 ↔ Bracket (15275A53):13
- Mate:278: BottomBasePlate_Rev2:1 ↔ Bracket (15275A53):13
- Mate:279: Base_Master_Rev2:1 ↔ Bracket (15275A53):13
- Mate:280: Base_Master_Rev2:1 ↔ Bracket (15275A53)_LeftCut:4
- Mate:281: BottomBasePlate_Rev2:1 ↔ Bracket (15275A53)_LeftCut:4
- Mate:282: Base_Master_Rev2:1 ↔ Bracket (15275A53)_LeftCut:4
- Mate:283: BottomBasePlate_Rev2:1 ↔ Bolted Connection:71
- Mate:284: BottomBasePlate_Rev2:1 ↔ Bolted Connection:71
- Mate:285: BottomBasePlate_Rev2:1 ↔ Bolted Connection:72
- Mate:286: BottomBasePlate_Rev2:1 ↔ Bolted Connection:72
- Mate:287: BottomBasePlate_Rev2:1 ↔ Bolted Connection:73
- Mate:288: BottomBasePlate_Rev2:1 ↔ Bolted Connection:73
- Mate:289: BottomBasePlate_Rev2:1 ↔ Bolted Connection:74
- Mate:290: BottomBasePlate_Rev2:1 ↔ Bolted Connection:74
- Mate:291: BottomBasePlate_Rev2:1 ↔ Bolted Connection:75
- Mate:292: BottomBasePlate_Rev2:1 ↔ Bolted Connection:75
- Mate:293: BottomBasePlate_Rev2:1 ↔ Bolted Connection:76
- Mate:294: BottomBasePlate_Rev2:1 ↔ Bolted Connection:76
- Mate:295: BottomBasePlate_Rev2:1 ↔ Bolted Connection:77
- Mate:296: BottomBasePlate_Rev2:1 ↔ Bolted Connection:77
- Mate:297: BottomBasePlate_Rev2:1 ↔ Bolted Connection:78
- Mate:298: BottomBasePlate_Rev2:1 ↔ Bolted Connection:78
- Mate:299: BottomBasePlate_Rev2:1 ↔ Bolted Connection:79
- Mate:300: BottomBasePlate_Rev2:1 ↔ Bolted Connection:79
- Mate:301: BottomBasePlate_Rev2:1 ↔ Bolted Connection:80
- Mate:302: BottomBasePlate_Rev2:1 ↔ Bolted Connection:80
- Mate:303: BottomBasePlate_Rev2:1 ↔ Bolted Connection:81
- Mate:304: BottomBasePlate_Rev2:1 ↔ Bolted Connection:81
- Mate:305: Base_Master_Rev2:1 ↔ Bolted Connection:82
- Mate:306: Base_Master_Rev2:1 ↔ Bolted Connection:82
- Mate:307: Base_Master_Rev2:1 ↔ Bolted Connection:83
- Mate:308: Base_Master_Rev2:1 ↔ Bolted Connection:83
- Mate:309: Base_Master_Rev2:1 ↔ Bolted Connection:84
- Mate:310: Base_Master_Rev2:1 ↔ Bolted Connection:84
- Mate:311: Base_Master_Rev2:1 ↔ Bolted Connection:85
- Mate:312: Base_Master_Rev2:1 ↔ Bolted Connection:85
- Mate:313: Base_Master_Rev2:1 ↔ Bolted Connection:86
- Mate:314: Base_Master_Rev2:1 ↔ Bolted Connection:86
- Mate:315: Base_Master_Rev2:1 ↔ Bolted Connection:87
- Mate:316: Base_Master_Rev2:1 ↔ Bolted Connection:87
